# Autodesk Inventor assembly: 組合窗_2_MIR6
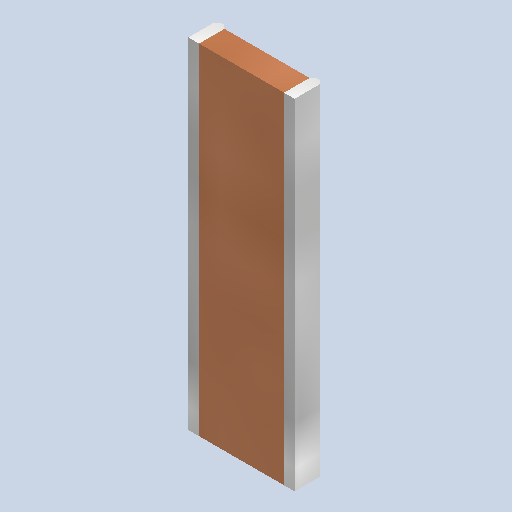
[picture p0: Inventor's stored thumbnail of the model, 512x512]
Saved by Autodesk Inventor 2024.2 (Build 282272000, 272)
## iProperties
Created: 2024-06-02
Part Number: 組合窗_2_MIR6
Document SubType Name: Assembly
Designer: User
Author: User
## Documents named in this file (3)
- C:\Users\User\OneDrive - 國立中山大學\桌面\創客基礎\final_project\mirror\組合窗_2_MIR6.iam
- C:\Users\User\OneDrive - 國立中山大學\桌面\創客基礎\final_project\mirror\窗_MIR13.ipt
- C:\Users\User\OneDrive - 國立中山大學\桌面\創客基礎\final_project\mirror\窗側柱_MIR13.ipt
## Components (3 placed, 2 different names)
1. 窗_MIR13:1 — 齊平:4, 齊平:3, 貼合:2, 齊平:2, 齊平:1, 貼合:1
2. 窗側柱_MIR13:1 — 齊平:4, 齊平:3, 貼合:2
3. 窗側柱_MIR13:2 — 齊平:2, 齊平:1, 貼合:1
## Relationships (6: Flush 4, Mate 2)
- 齊平:4 [Flush]: 窗_MIR13:1 ↔ 窗側柱_MIR13:1
- 齊平:3 [Flush]: 窗_MIR13:1 ↔ 窗側柱_MIR13:1
- 貼合:2 [Mate]: 窗_MIR13:1 ↔ 窗側柱_MIR13:1
- 齊平:2 [Flush]: 窗_MIR13:1 ↔ 窗側柱_MIR13:2
- 齊平:1 [Flush]: 窗_MIR13:1 ↔ 窗側柱_MIR13:2
- 貼合:1 [Mate]: 窗_MIR13:1 ↔ 窗側柱_MIR13:2
